# Autodesk Inventor assembly: 775pro_2_Female
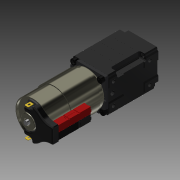
[picture p0: Inventor's stored thumbnail of the model, 180x180]
Saved by Autodesk Inventor 2021 (Build 250183000, 183)
## iProperties
Created: 2018-08-19
Part Number: 775pro_2_Female
Document SubType Name: Assembly
Designer: Rafi
Mass: 1123.04 g
Surface Area: 1203.25 cm^2
Volume: 285.054 cm^3
Density: 3.93975 g/cm^3
Author: Rafi
## Documents named in this file (8)
- D:\FIRST\FRC\1369\CollabPartsLib\Motors\Versaplanetary\VersaPlanetary\775pro, 2 Stages, Female Output.iam
- C:\Users\Cal\Desktop\FIRST\FRC\6814 Ellipse\Ellipse Design\Ellipse Parts Library\Gearboxes\Planetary Gearboxes\V2 Stages\V2 Output Stage.iam
- D:\FIRST\FRC\1369\CollabPartsLib\Motors\Versaplanetary\Intermediate Stages\Ring Gear.ipt
- C:\Users\Cal\Desktop\FIRST\FRC\6814 Ellipse\Ellipse Design\Ellipse Parts Library\Gearboxes\Planetary Gearboxes\V2 Stages\V2 Input Stage.iam
- D:\FIRST\FRC\1369\CollabPartsLib\Motors\Versaplanetary\Screws\8-32 x 2.25in Screw.ipt
- D:\FIRST\FRC\1369\CollabPartsLib\Motors\Versaplanetary\V2 Stages\V2 Input Stage\VP 775pro Input.iam
- D:\FIRST\FRC\1369\CollabPartsLib\Motors\Versaplanetary\VersaPlanetary.iam
- D:\FIRST\FRC\1369\CollabPartsLib\Motors\Versaplanetary\V2 Stages\V2 Output Stage\VP V2 Output Stage Female.iam
## Components (6 placed, 5 different names)
1. VP V2 Output Stage Female:1 [sub-assembly] — Insert:1, Flush:3, Flush:6, 2StageBasicInputMate2
2. Ring Gear 1 — Insert:1, Insert:2, Flush:1, Flush:3
3. Ring Gear 2 — Insert:2, Flush:1, Flush:6, 2StageBasicInputMate1
4. VP 775pro Input:1 [sub-assembly] — 2StageBasicInputMate1, 2StageBasicInputMate2, Insert:10, Insert:11
5. 8-32 x 2.25in Screw:1 — Insert:10
6. 8-32 x 2.25in Screw:2 — Insert:11
## Relationships (9: Insert 5, Flush 4)
- Insert:1: VP V2 Output Stage Female:1 ↔ Ring Gear 1
- Insert:2: Ring Gear 1 ↔ Ring Gear 2
- Flush:1: Ring Gear 1 ↔ Ring Gear 2
- Flush:3: VP V2 Output Stage Female:1 ↔ Ring Gear 1
- Flush:6: VP V2 Output Stage Female:1 ↔ Ring Gear 2
- 2StageBasicInputMate1 [Insert]: Ring Gear 2 ↔ VP 775pro Input:1
- 2StageBasicInputMate2 [Flush]: VP V2 Output Stage Female:1 ↔ VP 775pro Input:1
- Insert:10: VP 775pro Input:1 ↔ 8-32 x 2.25in Screw:1
- Insert:11: VP 775pro Input:1 ↔ 8-32 x 2.25in Screw:2
